# Autodesk Inventor assembly: Robot Assembly
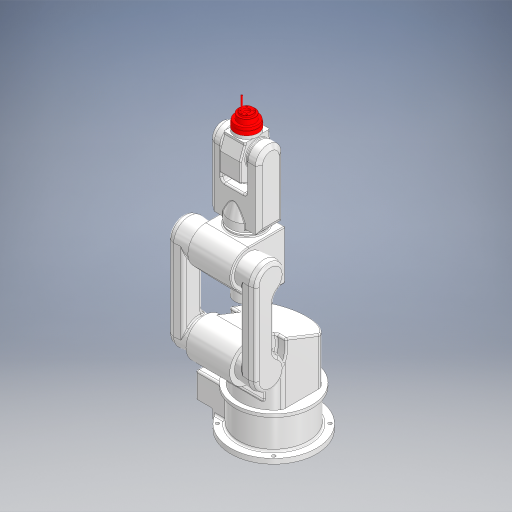
[picture p0: Inventor's stored thumbnail of the model, 512x512]
Saved by Autodesk Inventor 2024 (Build 280153000, 153)
## iProperties
Created: 2004-10-04
Part Number: Robot Assembly
Document SubType Name: Assembly
Designer: SSimmons
Sending System: SolidWorks 2017
Last Author: fdefersh
Last Saved: 2018-03-08
Author: SSimmons
## Documents named in this file (9)
- C:\Shared\alex-bartella-schoolwork\4z03\Week 9\STEP\CE-9.2.1 Pack and go\Robot Assembly.iam
- C:\Shared\alex-bartella-schoolwork\4z03\Week 9\STEP\CE-9.2.1 Pack and go\robot_base_&.ipt
- C:\Shared\alex-bartella-schoolwork\4z03\Week 9\STEP\CE-9.2.1 Pack and go\robot_lower_axis_&.ipt
- C:\Shared\alex-bartella-schoolwork\4z03\Week 9\STEP\CE-9.2.1 Pack and go\robot_arm_right_&.ipt
- C:\Shared\alex-bartella-schoolwork\4z03\Week 9\STEP\CE-9.2.1 Pack and go\robot_arm_left_&.ipt
- C:\Shared\alex-bartella-schoolwork\4z03\Week 9\STEP\CE-9.2.1 Pack and go\robot_upper_axis_&.ipt
- C:\Shared\alex-bartella-schoolwork\4z03\Week 9\STEP\CE-9.2.1 Pack and go\robot_forearm_&.ipt
- C:\Shared\alex-bartella-schoolwork\4z03\Week 9\STEP\CE-9.2.1 Pack and go\robot_wrist_&.ipt
- C:\Shared\alex-bartella-schoolwork\4z03\Week 9\STEP\CE-9.2.1 Pack and go\robot_flange_&.ipt
## Components (8 placed, 8 different names)
1. robot_base_&:1 — Mate:1, Mate:2, Angle:1
2. robot_lower_axis_&:1 — Mate:1, Mate:2, Mate:3, Mate:4, Angle:1, Mate:5, Mate:6, Angle:2
3. robot_arm_right_&:1 — Mate:4, Mate:5, Mate:7, Mate:9, Angle:2, Angle:3
4. robot_arm_left_&:1 — Mate:3, Mate:6, Mate:8
5. robot_upper_axis_&:1 — Mate:7, Mate:8, Mate:9, Mate:10, Angle:3, Angle:4, Mate:15
6. robot_forearm_&:1 — Mate:10, Mate:11, Mate:14, Angle:4, Mate:15, Angle:5
7. robot_wrist_&:1 — Mate:11, Mate:12, Mate:13, Mate:14, Angle:5, Angle:6
8. robot_flange_&:1 — Mate:12, Mate:13, Angle:6
## Relationships (21: Mate 15, Angle 6)
- Mate:1: robot_base_&:1 ↔ robot_lower_axis_&:1
- Mate:2: robot_base_&:1 ↔ robot_lower_axis_&:1
- Mate:3: robot_lower_axis_&:1 ↔ robot_arm_left_&:1
- Mate:4: robot_lower_axis_&:1 ↔ robot_arm_right_&:1
- Angle:1 (0 deg): robot_base_&:1 ↔ robot_lower_axis_&:1
- Mate:5: robot_lower_axis_&:1 ↔ robot_arm_right_&:1
- Mate:6: robot_lower_axis_&:1 ↔ robot_arm_left_&:1
- Mate:7: robot_arm_right_&:1 ↔ robot_upper_axis_&:1
- Mate:8: robot_arm_left_&:1 ↔ robot_upper_axis_&:1
- Mate:9: robot_arm_right_&:1 ↔ robot_upper_axis_&:1
- Mate:10: robot_upper_axis_&:1 ↔ robot_forearm_&:1
- Mate:11: robot_forearm_&:1 ↔ robot_wrist_&:1
- Mate:12: robot_wrist_&:1 ↔ robot_flange_&:1
- Mate:13: robot_wrist_&:1 ↔ robot_flange_&:1
- Mate:14: robot_forearm_&:1 ↔ robot_wrist_&:1
- Angle:2 (0 deg): robot_lower_axis_&:1 ↔ robot_arm_right_&:1
- Angle:3 (180 deg): robot_arm_right_&:1 ↔ robot_upper_axis_&:1
- Angle:4 (0 deg): robot_upper_axis_&:1 ↔ robot_forearm_&:1
- Mate:15 (5 mm): robot_upper_axis_&:1 ↔ robot_forearm_&:1
- Angle:5 (0 deg): robot_forearm_&:1 ↔ robot_wrist_&:1
- Angle:6 (0 deg): robot_wrist_&:1 ↔ robot_flange_&:1
